# Autodesk Inventor assembly: PowerDistroAssembly
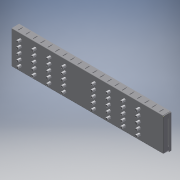
[picture p0: Inventor's stored thumbnail of the model, 180x180]
Saved by Autodesk Inventor 2018 (Build 220112000, 112)
## iProperties
Created: 2018-04-20
Part Number: PowerDistroAssembly
Document SubType Name: Assembly
Designer: Rich
Author: Rich
## Documents named in this file (7)
- C:\Users\Rich\development\UWaterloo\power-distro.git\SolidModels\PowerDistroAssembly.iam
- C:\Users\Rich\development\UWaterloo\power-distro.git\SolidModels\power_distro_pcb_RevB.ipt
- C:\Users\Rich\development\UWaterloo\power-distro.git\SolidModels\Enclosure_RevB.ipt
- C:\Users\Rich\development\UWaterloo\power-distro.git\SolidModels\rcj-021.ipt
- C:\Users\Rich\development\UWaterloo\power-distro.git\SolidModels\Enclosure_RevB_Bottom.ipt
- C:\Users\Rich\development\UWaterloo\power-distro.git\SolidModels\keystone-PN1608-2.ipt
- C:\Users\Rich\development\UWaterloo\power-distro.git\SolidModels\AAVID_7106.ipt
## Components (46 placed, 6 different names)
1. power_distro_pcb_RevB:1 — Mate:1, Mate:2, Mate:3, Mate:4, Angle:1, Mate:12, Mate:13, Mate:14, Mate:15
2. Enclosure_RevB:1 — Mate:5, Mate:6, Mate:7
3. Enclosure_RevB_Bottom:1 — Mate:8, Mate:9, Mate:10, Mate:11
4. keystone-PN1608-2:1 — Mate:8, Mate:9, Mate:12, Mate:13
5. keystone-PN1608-2:2 — Mate:10, Mate:11, Mate:14
6. AAVID_7106:1 — Mate:15
7. rcj-021:1 — Mate:4, Angle:1, Mate:7
8. rcj-021:2
9. rcj-021:3
10. rcj-021:4
11. rcj-021:5
12. rcj-021:6
13. rcj-021:7
14. rcj-021:8
15. rcj-021:9
16. rcj-021:10
17. rcj-021:11
18. rcj-021:12
19. rcj-021:13
20. rcj-021:14
21. rcj-021:15
22. rcj-021:16
23. rcj-021:17
24. rcj-021:18
25. rcj-021:19
26. rcj-021:20
27. rcj-021:21
28. rcj-021:22
29. rcj-021:23
30. rcj-021:24
31. rcj-021:25
32. rcj-021:26
33. rcj-021:27
34. rcj-021:28
35. rcj-021:29
36. rcj-021:30
37. rcj-021:31
38. rcj-021:32
39. rcj-021:33
40. rcj-021:34
41. rcj-021:35 — Mate:5
42. rcj-021:36
43. rcj-021:37
44. rcj-021:38
45. rcj-021:39
46. rcj-021:40 — Mate:6
## Component patterns: (2 elements), (20 elements, first: rcj-021:1), Component Pattern 1:2 (20 elements)
## Relationships (16: Mate 15, Angle 1)
- Mate:1: power_distro_pcb_RevB:1
- Mate:2: power_distro_pcb_RevB:1
- Mate:3: power_distro_pcb_RevB:1
- Mate:4: power_distro_pcb_RevB:1 ↔ rcj-021:1
- Angle:1 (0 deg): power_distro_pcb_RevB:1 ↔ rcj-021:1
- Mate:5: Enclosure_RevB:1 ↔ rcj-021:35
- Mate:6: Enclosure_RevB:1 ↔ rcj-021:40
- Mate:7: Enclosure_RevB:1 ↔ rcj-021:1
- Mate:8: Enclosure_RevB_Bottom:1 ↔ keystone-PN1608-2:1
- Mate:9: Enclosure_RevB_Bottom:1 ↔ keystone-PN1608-2:1
- Mate:10: Enclosure_RevB_Bottom:1 ↔ keystone-PN1608-2:2
- Mate:11: Enclosure_RevB_Bottom:1 ↔ keystone-PN1608-2:2
- Mate:12: power_distro_pcb_RevB:1 ↔ keystone-PN1608-2:1
- Mate:13: power_distro_pcb_RevB:1 ↔ keystone-PN1608-2:1
- Mate:14: power_distro_pcb_RevB:1 ↔ keystone-PN1608-2:2
- Mate:15: power_distro_pcb_RevB:1 ↔ AAVID_7106:1
